# Autodesk Inventor assembly: Base Assembly
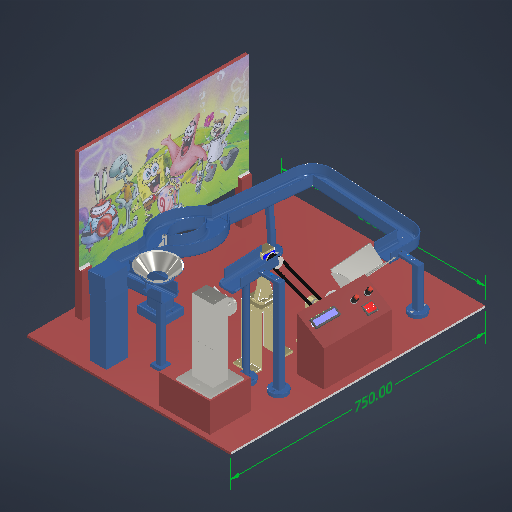
[picture p0: Inventor's stored thumbnail of the model, 512x512]
Saved by Autodesk Inventor 2026.2 (Build 302298010, 298A)
## iProperties
Created: 2026-04-15
Part Number: Base Assembly
Document SubType Name: Assembly
Designer: lenovo
Author: lenovo
## Documents named in this file (15)
- F:\Semester 4\Basics of Mechatronics\Final\Base Assembly.iam
- F:\Semester 4\Basics of Mechatronics\Final\Base.ipt
- F:\Semester 4\Basics of Mechatronics\Final\SORTING Assembly.iam
- F:\Semester 4\Basics of Mechatronics\Final\SHOOTING Assembly.0002.iam
- F:\Semester 4\Basics of Mechatronics\Final\Stand of Shooting.ipt
- F:\Semester 4\Basics of Mechatronics\Final\Housing of Buttons & LCD.ipt
- F:\Semester 4\Basics of Mechatronics\Final\Lifting Mechanism.iam
- F:\Semester 4\Basics of Mechatronics\Final\Path from Lifting to Shooting.ipt
- F:\Semester 4\Basics of Mechatronics\Final\Stand of theme.ipt
- F:\Semester 4\Basics of Mechatronics\Final\Part1.ipt
- F:\Semester 4\Basics of Mechatronics\Final\LCD_1602\LCD_1602\LCD_1602.ipt
- F:\Semester 4\Basics of Mechatronics\Final\PushButtonSwitch\PushButtonSwitch\PushButtonSwitch.ipt
- F:\Semester 4\Basics of Mechatronics\Final\KCD4\KCD4\KCD4.ipt
- F:\Semester 4\Basics of Mechatronics\Final\IR_LM393_pin.ipt
- F:\Semester 4\Basics of Mechatronics\Final\Storage Assembly.iam
## Components (18 placed, 14 different names)
1. Base:1 — Mate:3, Mate:5, Mate:10, Mate:12, Mate:14, Mate:17, Mate:34
2. SHOOTING Assembly:1 [sub-assembly] — Mate:4
3. Stand of Shooting:1 — Mate:3, Mate:4, Mate:18
4. SORTING Assembly:1 [sub-assembly] — Mate:5, Mate:30, Mate:32
5. Housing of Buttons & LCD:1 — Mate:10, Mate:20, Mate:21, Mate:22, Mate:23, Mate:24, Mate:25, Mate:26, Mate:27, Mate:28, Mate:29, Mate:31
6. Lifting Mechanism:1 [sub-assembly] — Mate:12
7. Path from Lifting to Shooting:1 — Mate:14, Mate:33
8. Stand of theme:1 — Mate:17
9. Part1:1 — Mate:18
10. LCD_1602:1 — Mate:20, Mate:21, Mate:22
11. PushButtonSwitch:2 — Mate:23, Mate:26
12. PushButtonSwitch:3 — Mate:24, Mate:25
13. KCD4:3 — Mate:27, Mate:28, Mate:29
14. IR_LM393_pin:1 — Mate:30
15. IR_LM393_pin:3 — Mate:32
16. IR_LM393_pin:4 — Mate:31
17. IR_LM393_pin:5 — Mate:33
18. Storage Assembly:1 [sub-assembly] — Mate:34
## Relationships (23: Mate 23)
- Mate:3: Base:1 ↔ Stand of Shooting:1
- Mate:4: SHOOTING Assembly:1 ↔ Stand of Shooting:1
- Mate:5: Base:1 ↔ SORTING Assembly:1
- Mate:10: Base:1 ↔ Housing of Buttons & LCD:1
- Mate:12: Base:1 ↔ Lifting Mechanism:1
- Mate:14: Base:1 ↔ Path from Lifting to Shooting:1
- Mate:17: Base:1 ↔ Stand of theme:1
- Mate:18: Stand of Shooting:1 ↔ Part1:1
- Mate:20: Housing of Buttons & LCD:1 ↔ LCD_1602:1
- Mate:21: Housing of Buttons & LCD:1 ↔ LCD_1602:1
- Mate:22: Housing of Buttons & LCD:1 ↔ LCD_1602:1
- Mate:23: Housing of Buttons & LCD:1 ↔ PushButtonSwitch:2
- Mate:24: Housing of Buttons & LCD:1 ↔ PushButtonSwitch:3
- Mate:25: Housing of Buttons & LCD:1 ↔ PushButtonSwitch:3
- Mate:26: Housing of Buttons & LCD:1 ↔ PushButtonSwitch:2
- Mate:27: Housing of Buttons & LCD:1 ↔ KCD4:3
- Mate:28: Housing of Buttons & LCD:1 ↔ KCD4:3
- Mate:29: Housing of Buttons & LCD:1 ↔ KCD4:3
- Mate:30: SORTING Assembly:1 ↔ IR_LM393_pin:1
- Mate:31: Housing of Buttons & LCD:1 ↔ IR_LM393_pin:4
- Mate:32: SORTING Assembly:1 ↔ IR_LM393_pin:3
- Mate:33: Path from Lifting to Shooting:1 ↔ IR_LM393_pin:5
- Mate:34: Base:1 ↔ Storage Assembly:1
